# Autodesk Inventor assembly: servomotorFakeShast
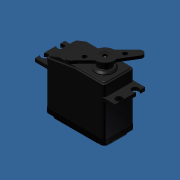
[picture p0: Inventor's stored thumbnail of the model, 180x180]
Saved by Autodesk Inventor 2014 (Build 180170000, 170)
## iProperties
Created: 2014-04-17
Part Number: servomotorFakeShast
Document SubType Name: Assembly
Designer: Lefo
Author: Lefo
## Documents named in this file (5)
- C:\Users\Lefo\Documents\Inventor\academy\servo power HD1501MG\servomotorFakeShast.iam
- C:\Users\Lefo\Documents\Inventor\academy\servo power HD1501MG\carcaza servo power modificado.ipt
- C:\Users\Lefo\Documents\Inventor\academy\tapaServoEjeFalso.ipt
- C:\Users\Lefo\Documents\Inventor\academy\servo power HD1501MG\pinhon servo.ipt
- C:\Users\Lefo\Documents\Inventor\academy\servo power HD1501MG\acople estrella2 servo.ipt
## Components (4 placed, 4 different names)
1. carcaza servo power modificado:1 — Mate:1, Flush:1, Flush:2, Insert:1
2. tapaServoEjeFalso:1 — Mate:1, Flush:1, Flush:2
3. pinhon servo:1 — Insert:1, Insert:2
4. acople estrella2 servo:1 — Insert:2
## Relationships (5: Flush 2, Insert 2, Mate 1)
- Mate:1: carcaza servo power modificado:1 ↔ tapaServoEjeFalso:1
- Flush:1 (-0.05 mm): carcaza servo power modificado:1 ↔ tapaServoEjeFalso:1
- Flush:2 (-0.15 mm): carcaza servo power modificado:1 ↔ tapaServoEjeFalso:1
- Insert:1: carcaza servo power modificado:1 ↔ pinhon servo:1
- Insert:2: pinhon servo:1 ↔ acople estrella2 servo:1
